# Autodesk Inventor assembly: PILLARSCELLCASE21700ASSEMBLY
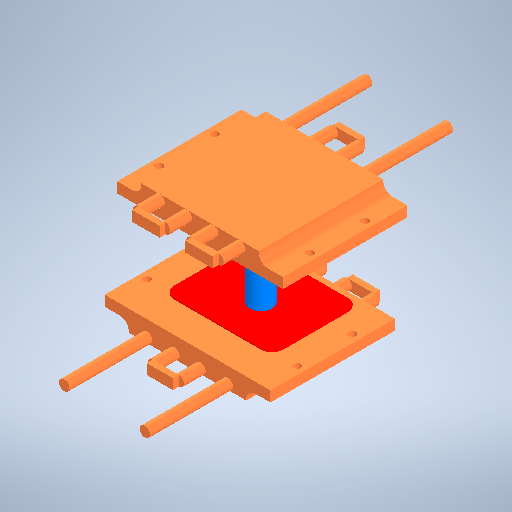
[picture p0: Inventor's stored thumbnail of the model, 512x512]
Saved by Autodesk Inventor 2025.2 (Build 292293000, 293)
## iProperties
Created: 2025-06-10
Part Number: PILLARSCELLCASE21700ASSEMBLY
Document SubType Name: Assembly
Designer: cbast
Author: cbast
## Documents named in this file (4)
- C:\Users\cbast\OneDrive\Documents\GitHub\Smart-Pack-for-Advanced-Research-and-Control\variations\Camden\V0.2\PILLARSCELLCASE21700ASSEMBLY.iam
- C:\Users\cbast\OneDrive\Documents\GitHub\Smart-Pack-for-Advanced-Research-and-Control\variations\Camden\V0.1\21700(Blue).ipt
- C:\Users\cbast\OneDrive\Documents\GitHub\Smart-Pack-for-Advanced-Research-and-Control\variations\Camden\V0.1\343thermalpad.ipt
- C:\Users\cbast\OneDrive\Documents\GitHub\Smart-Pack-for-Advanced-Research-and-Control\variations\Camden\V0.1\cooling plate.ipt
## Components (5 placed, 3 different names)
1. 21700(Blue):1 — Mate:1, Mate:2
2. 343thermalpad:1 — Mate:2, Mate:3
3. 343thermalpad:2 — Mate:1, Mate:4
4. cooling plate:1 — Mate:3
5. cooling plate:2 — Mate:4
## Relationships (4: Mate 4)
- Mate:1: 21700(Blue):1 ↔ 343thermalpad:2
- Mate:2: 21700(Blue):1 ↔ 343thermalpad:1
- Mate:3: 343thermalpad:1 ↔ cooling plate:1
- Mate:4: 343thermalpad:2 ↔ cooling plate:2
